# Autodesk Inventor assembly: bonsai
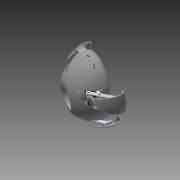
[picture p0: Inventor's stored thumbnail of the model, 180x180]
Saved by Autodesk Inventor 2014 (Build 180170000, 170)
## iProperties
Created: 2015-05-23
Part Number: bonsai
Document SubType Name: Assembly
Designer: Hideyuki Takei
Author: Hideyuki Takei
## Documents named in this file (16)
- C:\Users\hide\Desktop\soth-bonsai\cad\body-asm\bonsai.iam
- C:\Users\hide\Desktop\soth-bonsai\cad\front-left.iam
- C:\Users\hide\Desktop\soth-bonsai\cad\front-right.iam
- C:\Users\hide\Desktop\soth-bonsai\cad\body-asm\body.ipt
- C:\Users\hide\Desktop\soth-bonsai\cad\RS304md-simple.ipt
- C:\Users\hide\Desktop\soth-bonsai\cad\RS304MD-ServoHorn.ipt
- C:\Users\hide\Desktop\soth-bonsai\cad\gear\servo-gear.ipt
- C:\Users\hide\Desktop\soth-bonsai\cad\gear\small-free-gear.ipt
- C:\Users\hide\Desktop\soth-bonsai\cad\gear\big-free-gear.ipt
- C:\Users\hide\Desktop\soth-bonsai\cad\gear\leg-gear.ipt
- C:\Users\hide\Desktop\soth-bonsai\cad\body-asm\body-cover.ipt
- C:\Users\hide\Desktop\soth-bonsai\cad\exoskeletal\exoskeletal-body.ipt
- C:\Users\hide\Desktop\soth-bonsai\cad\exoskeletal\front-right-leg.ipt
- C:\Users\hide\Desktop\soth-bonsai\cad\exoskeletal\front-left-leg.ipt
- C:\Users\hide\Desktop\soth-bonsai\cad\exoskeletal\back-right-leg.ipt
- C:\Users\hide\Desktop\soth-bonsai\cad\exoskeletal\back-left-leg.ipt
## Components (22 placed, 15 different names)
1. front-left:1 [sub-assembly] — メイト:5, メイト:13, メイト:33, メイト:34, メイト:48, メイト:49, メイト:50
2. front-left:2 [sub-assembly] — メイト:1, メイト:11, メイト:35, メイト:36, メイト:51, メイト:52, メイト:53
3. front-right:1 [sub-assembly] — メイト:6, メイト:12, メイト:30, メイト:31, メイト:45, メイト:46, メイト:47
4. front-right:2 [sub-assembly] — メイト:3, メイト:10, メイト:37, メイト:38, メイト:54, メイト:55, メイト:56
5. body:1 — メイト:1, メイト:3, メイト:5, メイト:6, メイト:9, メイト:10, メイト:11, メイト:12, メイト:13, メイト:14, メイト:15, メイト:16, メイト:22, メイト:23, メイト:24, メイト:25, メイト:26, メイト:27, メイト:28, メイト:29, メイト:32, メイト:39, メイト:40, メイト:41, メイト:42
6. RS304md-simple:1 — メイト:9, メイト:14, メイト:15, メイト:16, メイト:17, メイト:18
7. RS304MD-ServoHorn:1 — メイト:17, メイト:18, メイト:19, メイト:20, メイト:21
8. servo-gear:1 — メイト:19, メイト:20, メイト:21
9. small-free-gear:1 — メイト:23, メイト:25
10. small-free-gear:2 — メイト:22, メイト:24
11. big-free-gear:1 — メイト:27, メイト:28
12. big-free-gear:2 — メイト:26, メイト:29
13. leg-gear:1 — メイト:30, メイト:31, メイト:32
14. leg-gear:2 — メイト:33, メイト:34
15. leg-gear:3 — メイト:35, メイト:36
16. leg-gear:4 — メイト:37, メイト:38
17. body-cover:1 — メイト:39, メイト:40, メイト:41, メイト:43, メイト:44
18. exoskeletal-body:1 — メイト:42, メイト:43, メイト:44
19. front-right-leg:1 — メイト:45, メイト:46, メイト:47
20. front-left-leg:1 — メイト:48, メイト:49, メイト:50
21. back-right-leg:1 — メイト:51, メイト:52, メイト:53
22. back-left-leg:1 — メイト:54, メイト:55, メイト:56
## Relationships (52: Mate 52)
- メイト:1 [Mate]: front-left:2 ↔ body:1
- メイト:3 [Mate]: front-right:2 ↔ body:1
- メイト:5 [Mate]: front-left:1 ↔ body:1
- メイト:6 [Mate]: front-right:1 ↔ body:1
- メイト:9 [Mate]: body:1 ↔ RS304md-simple:1
- メイト:10 [Mate]: front-right:2 ↔ body:1
- メイト:11 [Mate]: front-left:2 ↔ body:1
- メイト:12 [Mate]: front-right:1 ↔ body:1
- メイト:13 [Mate]: front-left:1 ↔ body:1
- メイト:14 [Mate]: body:1 ↔ RS304md-simple:1
- メイト:15 [Mate]: body:1 ↔ RS304md-simple:1
- メイト:16 [Mate]: body:1 ↔ RS304md-simple:1
- メイト:17 [Mate]: RS304md-simple:1 ↔ RS304MD-ServoHorn:1
- メイト:18 [Mate]: RS304md-simple:1 ↔ RS304MD-ServoHorn:1
- メイト:19 [Mate]: RS304MD-ServoHorn:1 ↔ servo-gear:1
- メイト:20 [Mate]: RS304MD-ServoHorn:1 ↔ servo-gear:1
- メイト:21 [Mate]: RS304MD-ServoHorn:1 ↔ servo-gear:1
- メイト:22 [Mate]: body:1 ↔ small-free-gear:2
- メイト:23 [Mate]: body:1 ↔ small-free-gear:1
- メイト:24 [Mate]: body:1 ↔ small-free-gear:2
- メイト:25 [Mate]: body:1 ↔ small-free-gear:1
- メイト:26 [Mate]: body:1 ↔ big-free-gear:2
- メイト:27 [Mate]: body:1 ↔ big-free-gear:1
- メイト:28 [Mate]: body:1 ↔ big-free-gear:1
- メイト:29 [Mate]: body:1 ↔ big-free-gear:2
- メイト:30 [Mate]: front-right:1 ↔ leg-gear:1
- メイト:31 [Mate]: front-right:1 ↔ leg-gear:1
- メイト:32 [Mate]: body:1 ↔ leg-gear:1
- メイト:33 [Mate]: front-left:1 ↔ leg-gear:2
- メイト:34 [Mate]: front-left:1 ↔ leg-gear:2
- メイト:35 [Mate]: front-left:2 ↔ leg-gear:3
- メイト:36 [Mate]: front-left:2 ↔ leg-gear:3
- メイト:37 [Mate]: front-right:2 ↔ leg-gear:4
- メイト:38 [Mate]: front-right:2 ↔ leg-gear:4
- メイト:39 [Mate]: body:1 ↔ body-cover:1
- メイト:40 [Mate]: body:1 ↔ body-cover:1
- メイト:41 [Mate]: body:1 ↔ body-cover:1
- メイト:42 [Mate]: body:1 ↔ exoskeletal-body:1
- メイト:43 [Mate]: body-cover:1 ↔ exoskeletal-body:1
- メイト:44 [Mate]: body-cover:1 ↔ exoskeletal-body:1
- メイト:45 [Mate]: front-right:1 ↔ front-right-leg:1
- メイト:46 [Mate]: front-right:1 ↔ front-right-leg:1
- メイト:47 [Mate]: front-right:1 ↔ front-right-leg:1
- メイト:48 [Mate]: front-left:1 ↔ front-left-leg:1
- メイト:49 [Mate]: front-left:1 ↔ front-left-leg:1
- メイト:50 [Mate]: front-left:1 ↔ front-left-leg:1
- メイト:51 [Mate]: front-left:2 ↔ back-right-leg:1
- メイト:52 [Mate]: front-left:2 ↔ back-right-leg:1
- メイト:53 [Mate]: front-left:2 ↔ back-right-leg:1
- メイト:54 [Mate]: front-right:2 ↔ back-left-leg:1
- メイト:55 [Mate]: front-right:2 ↔ back-left-leg:1
- メイト:56 [Mate]: front-right:2 ↔ back-left-leg:1
